# Autodesk Inventor assembly: FlyWheelAssembly3
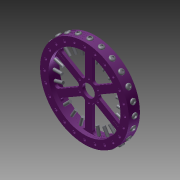
[picture p0: Inventor's stored thumbnail of the model, 180x180]
Saved by Autodesk Inventor 2012 (Build 160160000, 160)
## iProperties
Created: 2012-01-22
Part Number: FlyWheelAssembly3
Document SubType Name: Assembly
Designer: Logan
Author: Logan
## Documents named in this file (4)
- C:\Users\Logan\Desktop\FRC CAD Files\FlyWheelAssembly3.iam
- C:\Users\Logan\Desktop\team1885frc\Robot2012\Shooter\FlyWheelBase3.ipt
- C:\Users\Logan\Desktop\team1885frc\Robot2012\Shooter\ShooterWeight.ipt
- C:\Users\Logan\Desktop\team1885frc\Robot2012\Shooter\FlyWheelWeight.ipt
## Components (30 placed, 3 different names)
1. FlyWheelBase3:1 — Mate:1, Mate:2, Mate:3, Mate:7, Mate:8
2. FlyWheelBase3:2 — Mate:1, Mate:2, Mate:3, Mate:9, Mate:10, Mate:13, Mate:14
3. FlyWheelWeight:1 — Mate:5, Mate:6, Mate:7, Mate:8
4. FlyWheelWeight:2 — Mate:5, Mate:6
5. FlyWheelWeight:3 — Mate:9, Mate:10, Mate:11, Mate:12
6. FlyWheelWeight:4 — Mate:11, Mate:12
7. ShooterWeight:1 — Mate:13, Mate:14
8. ShooterWeight:2
9. ShooterWeight:3
10. ShooterWeight:4
11. ShooterWeight:5
12. ShooterWeight:6
13. ShooterWeight:7
14. ShooterWeight:8
15. ShooterWeight:9
16. ShooterWeight:10
17. ShooterWeight:11
18. ShooterWeight:12
19. ShooterWeight:13
20. ShooterWeight:14
21. ShooterWeight:15
22. ShooterWeight:16
23. ShooterWeight:17
24. ShooterWeight:18
25. ShooterWeight:19
26. ShooterWeight:20
27. ShooterWeight:21
28. ShooterWeight:22
29. ShooterWeight:23
30. ShooterWeight:24
## Component patterns: (24 elements, first: ShooterWeight:1)
## Relationships (13: Mate 13)
- Mate:1: FlyWheelBase3:1 ↔ FlyWheelBase3:2
- Mate:2: FlyWheelBase3:1 ↔ FlyWheelBase3:2
- Mate:3: FlyWheelBase3:1 ↔ FlyWheelBase3:2
- Mate:5: FlyWheelWeight:1 ↔ FlyWheelWeight:2
- Mate:6: FlyWheelWeight:1 ↔ FlyWheelWeight:2
- Mate:7: FlyWheelBase3:1 ↔ FlyWheelWeight:1
- Mate:8: FlyWheelBase3:1 ↔ FlyWheelWeight:1
- Mate:9: FlyWheelBase3:2 ↔ FlyWheelWeight:3
- Mate:10: FlyWheelBase3:2 ↔ FlyWheelWeight:3
- Mate:11: FlyWheelWeight:3 ↔ FlyWheelWeight:4
- Mate:12: FlyWheelWeight:3 ↔ FlyWheelWeight:4
- Mate:13: FlyWheelBase3:2 ↔ ShooterWeight:1
- Mate:14: FlyWheelBase3:2 ↔ ShooterWeight:1
